# Autodesk Inventor assembly: Baugruppe2
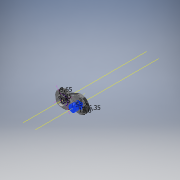
[picture p0: Inventor's stored thumbnail of the model, 180x180]
Saved by Autodesk Inventor 2018.3 (Build 223284000, 284)
## iProperties
Created: 2018-07-27
Part Number: Baugruppe2
Material: Generisch
Document SubType Name: Assembly
Designer: JochenAlt
Author: JochenAlt
## Documents named in this file (3)
- D:\Projects\FlowerPot\CAD\Beltdrive\BeltDriveConstruction.iam
- D:\Projects\FlowerPot\CAD\Beltdrive\Konstruktions-Assistent\Übertragung des Zahnriemens2.iam
- D:\Projects\FlowerPot\CAD\Beltdrive\BeltDriveConstruction\Konstruktions-Assistent\Übertragung des Zahnriemens1.iam
## Components (2 placed, 1 different names)
1. Übertragung des Zahnriemens:2 [sub-assembly] — Passend:4, Passend:6, Passend:7, Drehung:1, Passend:9
2. Übertragung des Zahnriemens:3 [sub-assembly] — Passend:6, Passend:8, Drehung:1, Passend:9
## Relationships (6: Mate 5, RelateRotation 1)
- Passend:4 [Mate]: Übertragung des Zahnriemens:2
- Passend:6 [Mate]: Übertragung des Zahnriemens:2 ↔ Übertragung des Zahnriemens:3
- Passend:7 [Mate]: Übertragung des Zahnriemens:2
- Passend:8 [Mate]: Übertragung des Zahnriemens:3
- Drehung:1 [RelateRotation] (1 ul): Übertragung des Zahnriemens:2 ↔ Übertragung des Zahnriemens:3
- Passend:9 [Mate] (1 mm): Übertragung des Zahnriemens:2 ↔ Übertragung des Zahnriemens:3
